# Autodesk Inventor assembly: ASY SLM 1110 MAIN FRAME
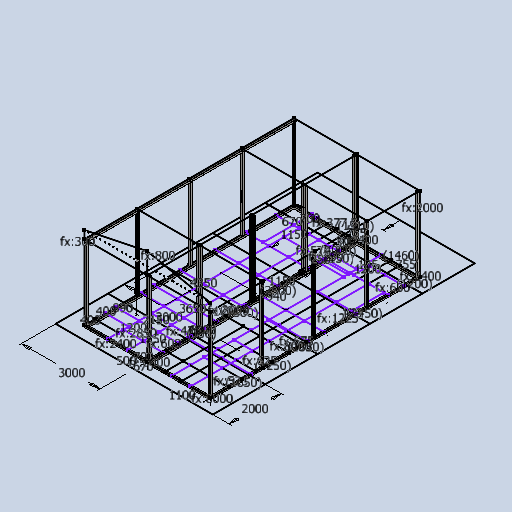
[picture p0: Inventor's stored thumbnail of the model, 512x512]
Saved by Autodesk Inventor 2025.3 (Build 293356030, 356C)
## iProperties
_SolveAssemblyDoc: Frame Generator Solve Assembly
_Version: 25.0.0
Created: 2025-12-15
Part Number: ASY SLM 1110 MAIN FRAME
Document SubType Name: Assembly
Designer: admin
Author: admin
## Documents named in this file (6)
- C:\Users\admin\Yandex.Disk\home pc\Inventor\SLM Salemal\ASY SLM 1110 MAIN FRAME.iam
- C:\Users\admin\Yandex.Disk\home pc\Inventor\SLM Salemal\ASY SLM 0110 left module.iam
- C:\Users\admin\Yandex.Disk\home pc\Inventor\SLM Salemal\Frame\ASY SLM 0120 right module.iam
- C:\Users\admin\Yandex.Disk\home pc\Inventor\SLM Salemal\PNS 1000 MAIN FRAME DIM.ipt
- C:\Users\admin\Yandex.Disk\home pc\Inventor\SLM Salemal\Frame\PNS-1100 FRAME Main sketch.ipt
- C:\Users\admin\Yandex.Disk\home pc\Inventor\SLM Salemal\ASY SLM 1110 MAIN FRAME\Frame\Frame 1765790796796.iam
## Components (5 placed, 5 different names)
1. ASY SLM 0110 left module:1 [sub-assembly] — Mate:1
2. ASY SLM 0120 right module:1 [sub-assembly]
3. PNS 1000 MAIN FRAME DIM:1
4. PNS-1100 FRAME Main sketch:1 — Mate:1
5. Frame 1765790796796:1 [sub-assembly]
## Relationships (2: WeldJoint 1, Mate 1)
- [WeldJoint]: ASY SLM 0110 left module:1 ↔ ASY SLM 0120 right module:1
- Mate:1: ASY SLM 0110 left module:1 ↔ PNS-1100 FRAME Main sketch:1
